# Autodesk Inventor assembly: Asem_Rev2
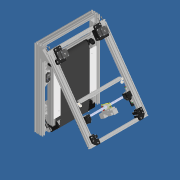
[picture p0: Inventor's stored thumbnail of the model, 180x180]
Saved by Autodesk Inventor 2020 (Build 240168000, 168)
## iProperties
Created: 2020-10-05
Part Number: Asem_Rev2
Document SubType Name: Assembly
Designer: magnarecta
Author: magnarecta
## Documents named in this file (20)
- D:\Document\Github\CoreXY_Laser\Model\Asem\Asem_Rev2.iam
- D:\Document\Github\CoreXY_Laser\Model\Asem\CoreXY_Unit_Asem.iam
- D:\Document\Github\CoreXY_Laser\Model\Parts\MISUMI\HFS5-2060-560_Autodesk_Inventor_2020_20201006\HFS5-2060-560.ipt
- D:\Document\Github\CoreXY_Laser\Model\Asem\Belt_Unit_Asem_Rev3.iam
- D:\Document\Github\CoreXY_Laser\Model\Parts\MISUMI\HFS5-2040-380_Autodesk_Inventor_2020_20201031\HFS5-2040-380.ipt
- D:\Document\Github\CoreXY_Laser\Model\Parts\MISUMI\HBLFSD5-SEC_Autodesk_Inventor_2020_20201031\AIS2020\HBLFSD5-SEC.iam
- D:\Document\Github\CoreXY_Laser\Model\Parts\MISUMI\HBLFSN5-SEC_Autodesk_Inventor_2020_20201031\AIS2020\HBLFSN5-SEC.iam
- D:\Document\Github\CoreXY_Laser\Model\Parts\MISUMI\HBLFSNF5-SEC_Autodesk_Inventor_2020_20201031\AIS2020\HBLFSNF5-SEC_b.iam
- D:\Document\Github\CoreXY_Laser\Model\Parts\Electrical_Components\mean-well-lrs-350-24-1.snapshot.3\meanwell_lrs-350-24_UPDATED.ipt
- D:\Document\Github\CoreXY_Laser\Model\Parts\Electrical_Components\BIGTREETECH_SKR_V1.4\BTT_SKR_V1.4 v13_TOP.iam
- D:\Document\Github\CoreXY_Laser\Model\Parts\Electrical_Components\ac-power-switch-assembly-1.snapshot.2\AC Power Switch Assy.iam
- D:\Document\Github\CoreXY_Laser\Model\Parts\Print_Parts\Rev2_Parts\Print_Parts_L1.ipt
- D:\Document\Github\CoreXY_Laser\Model\Parts\Electrical_Components\biqu-heat-bed-power-module-expansion-hot-bed-mos-tube-for-3d-printer-1.snapshot.2\BIQU-3D0109.iam
- D:\Document\Github\CoreXY_Laser\Model\Parts\Print_Parts\Rev2_Parts\Print_Parts_E2.ipt
- D:\Document\Github\CoreXY_Laser\Model\Parts\Electrical_Components\bigtreetech-tft-24-touchscreen-1.snapshot.2\BIGTREE_TFT24.iam
- D:\Document\Github\CoreXY_Laser\Model\Parts\Print_Parts\Rev2_Parts\Print_Parts_TFT.ipt
- D:\Document\Github\CoreXY_Laser\Model\Parts\Print_Parts\Print_Parts_V.ipt
- D:\Document\Github\CoreXY_Laser\Model\Parts\Print_Parts\Print_Parts_W.ipt
- D:\Document\Github\CoreXY_Laser\Model\Parts\Print_Parts\Print_Model\Controller_Unit\C_Unit_Cable_Holder_A.ipt
- D:\Document\Github\CoreXY_Laser\Model\Parts\Print_Parts\Print_Model\Controller_Unit\C_Unit_Cable_Holder_B.ipt
## Components (36 placed, 19 different names)
1. CoreXY_Unit_Asem:1 [sub-assembly] — フラッシュ:60, メイト:75, メイト:76
2. HFS5-2060-560:1 — フラッシュ:18, フラッシュ:19, Mate:16, Mate:17, Flush:28, Flush:29, Mate:18, Mate:25, Mate:32, Mate:33, Mate:45, Mate:49, Mate:61, メイト:77
3. HFS5-2060-560:2 — フラッシュ:18, フラッシュ:19, メイト:14, Flush:26, Flush:27, Mate:21, Mate:24, Mate:34, Mate:35, Mate:36, Flush:43, Mate:37, Mate:40, Mate:43, Mate:44, フラッシュ:60, フラッシュ:62, メイト:78, メイト:79, フラッシュ:63
4. Belt_Unit_Asem_Rev3:1 [sub-assembly] — メイト:14, Flush:38, Mate:51, Mate:52, Mate:53, Mate:54, Flush:51, Flush:53, Mate:59
5. HFS5-2040-380:1 — Mate:16, Flush:26, Flush:27, Mate:22, Mate:23, Flush:33, Flush:38, Mate:69, 角度:6, フラッシュ:64, メイト:83
6. HFS5-2040-380:2 — Mate:17, Flush:28, Flush:29, Mate:19, Mate:20, Flush:31, Mate:40, メイト:73
7. HBLFSD5-SEC:1 [sub-assembly] — Mate:18, Mate:19, Flush:30
8. HBLFSD5-SEC:2 [sub-assembly] — Mate:20, Mate:21, Flush:30, Flush:31
9. HBLFSD5-SEC:3 [sub-assembly] — Mate:22, Mate:25, Flush:32
10. HBLFSD5-SEC:4 [sub-assembly] — Mate:23, Mate:24, Flush:32, Flush:33
11. HBLFSN5-SEC:1 [sub-assembly] — Mate:33, Flush:40, Mate:50, Flush:49
12. HBLFSN5-SEC:2 [sub-assembly] — Mate:32, Flush:40, Flush:42, Flush:48, Mate:47
13. HBLFSN5-SEC:3 [sub-assembly] — Mate:34, Flush:41, Mate:38, Flush:45, Flush:47
14. HBLFSN5-SEC:4 [sub-assembly] — Mate:35, Flush:41, Flush:42, Mate:39, Flush:46
15. HFS5-2040-380:3 — Mate:36, Flush:43, Flush:44, Mate:38, Flush:45, Mate:41, Mate:48, Mate:50, Mate:56, Mate:57, Mate:59, メイト:73, メイト:84, フラッシュ:65, メイト:91, フラッシュ:67
16. HFS5-2040-380:4 — Mate:37, Flush:44, Mate:39, Mate:42, Mate:46, Mate:47, Mate:55, Mate:58, Mate:69, メイト:87
17. HBLFSN5-SEC:5 [sub-assembly] — Mate:45, Mate:46, Flush:48
18. HBLFSN5-SEC:6 [sub-assembly] — Mate:48, Mate:49, Flush:49
19. HBLFSN5-SEC:7 [sub-assembly] — Mate:41, Mate:43, Flush:47
20. HBLFSN5-SEC:8 [sub-assembly] — Mate:42, Mate:44, Flush:46
21. HBLFSNF5-SEC_b:1 [sub-assembly] — Mate:51, Mate:57, Flush:50, Flush:51
22. HBLFSNF5-SEC_b:2 [sub-assembly] — Mate:52, Mate:58, Flush:50
23. HBLFSNF5-SEC_b:3 [sub-assembly] — Mate:53, Mate:56, Flush:52, Flush:53
24. HBLFSNF5-SEC_b:4 [sub-assembly] — Mate:54, Mate:55, Flush:52
25. AC Power Switch Assy:1 [sub-assembly] — Mate:61, 挿入:3, 挿入:4
26. BIQU-3D0109:1 [sub-assembly] — 挿入:7, メイト:89
27. Print_Parts_L1:4 — メイト:75, メイト:76, フラッシュ:62, メイト:77, メイト:78
28. Print_Parts_E2:1 — メイト:79, フラッシュ:63, 挿入:3, 挿入:4
29. BIGTREE_TFT24:1 [sub-assembly] — メイト:80, メイト:81, メイト:82
30. Print_Parts_TFT:1 — メイト:80, メイト:81, メイト:82, 角度:6, フラッシュ:64, メイト:83
31. Print_Parts_V:1 — メイト:84, フラッシュ:65, メイト:85, 角度:7, 挿入:5, メイト:86, フラッシュ:66
32. meanwell_lrs-350-24_UPDATED:2 — メイト:85, 角度:7, 挿入:5
33. BTT_SKR_V1.4 v13_TOP:2 [sub-assembly] — 挿入:6, メイト:88
34. Print_Parts_W:2 — メイト:86, フラッシュ:66, メイト:87, 挿入:6, メイト:88, 挿入:7, メイト:89
35. C_Unit_Cable_Holder_A:1 — 挿入:8, メイト:92
36. C_Unit_Cable_Holder_B:1 — メイト:91, フラッシュ:67, 挿入:8, メイト:92
## Relationships (99: Mate 59, Flush 32, Insert 6, Angle 2)
- フラッシュ:18 [Flush]: HFS5-2060-560:1 ↔ HFS5-2060-560:2
- フラッシュ:19 [Flush]: HFS5-2060-560:1 ↔ HFS5-2060-560:2
- メイト:14 [Mate] (35 mm): HFS5-2060-560:2 ↔ Belt_Unit_Asem_Rev3:1
- Mate:16: HFS5-2060-560:1 ↔ HFS5-2040-380:1
- Flush:26: HFS5-2060-560:2 ↔ HFS5-2040-380:1
- Flush:27: HFS5-2060-560:2 ↔ HFS5-2040-380:1
- Mate:17: HFS5-2060-560:1 ↔ HFS5-2040-380:2
- Flush:28: HFS5-2060-560:1 ↔ HFS5-2040-380:2
- Flush:29: HFS5-2060-560:1 ↔ HFS5-2040-380:2
- Mate:18: HFS5-2060-560:1 ↔ HBLFSD5-SEC:1
- Mate:19: HFS5-2040-380:2 ↔ HBLFSD5-SEC:1
- Mate:20: HFS5-2040-380:2 ↔ HBLFSD5-SEC:2
- Mate:21: HFS5-2060-560:2 ↔ HBLFSD5-SEC:2
- Flush:30: HBLFSD5-SEC:1 ↔ HBLFSD5-SEC:2
- Flush:31: HFS5-2040-380:2 ↔ HBLFSD5-SEC:2
- Mate:22: HFS5-2040-380:1 ↔ HBLFSD5-SEC:3
- Mate:23: HFS5-2040-380:1 ↔ HBLFSD5-SEC:4
- Mate:24: HFS5-2060-560:2 ↔ HBLFSD5-SEC:4
- Mate:25: HFS5-2060-560:1 ↔ HBLFSD5-SEC:3
- Flush:32: HBLFSD5-SEC:3 ↔ HBLFSD5-SEC:4
- Flush:33: HFS5-2040-380:1 ↔ HBLFSD5-SEC:4
- Flush:38: Belt_Unit_Asem_Rev3:1 ↔ HFS5-2040-380:1
- Mate:32: HFS5-2060-560:1 ↔ HBLFSN5-SEC:2
- Mate:33: HFS5-2060-560:1 ↔ HBLFSN5-SEC:1
- Flush:40: HBLFSN5-SEC:1 ↔ HBLFSN5-SEC:2
- Mate:34: HFS5-2060-560:2 ↔ HBLFSN5-SEC:3
- Mate:35: HFS5-2060-560:2 ↔ HBLFSN5-SEC:4
- Flush:41: HBLFSN5-SEC:3 ↔ HBLFSN5-SEC:4
- Flush:42: HBLFSN5-SEC:2 ↔ HBLFSN5-SEC:4
- Mate:36: HFS5-2060-560:2 ↔ HFS5-2040-380:3
- Flush:43 (20 mm): HFS5-2060-560:2 ↔ HFS5-2040-380:3
- Mate:37: HFS5-2060-560:2 ↔ HFS5-2040-380:4
- Flush:44: HFS5-2040-380:3 ↔ HFS5-2040-380:4
- Mate:38: HBLFSN5-SEC:3 ↔ HFS5-2040-380:3
- Flush:45: HBLFSN5-SEC:3 ↔ HFS5-2040-380:3
- Mate:39: HBLFSN5-SEC:4 ↔ HFS5-2040-380:4
- Mate:40: HFS5-2060-560:2 ↔ HFS5-2040-380:2
- Mate:41: HFS5-2040-380:3 ↔ HBLFSN5-SEC:7
- Mate:42: HFS5-2040-380:4 ↔ HBLFSN5-SEC:8
- Mate:43: HFS5-2060-560:2 ↔ HBLFSN5-SEC:7
- Mate:44: HFS5-2060-560:2 ↔ HBLFSN5-SEC:8
- Flush:46: HBLFSN5-SEC:4 ↔ HBLFSN5-SEC:8
- Flush:47: HBLFSN5-SEC:3 ↔ HBLFSN5-SEC:7
- Mate:45: HFS5-2060-560:1 ↔ HBLFSN5-SEC:5
- Mate:46: HFS5-2040-380:4 ↔ HBLFSN5-SEC:5
- Flush:48: HBLFSN5-SEC:2 ↔ HBLFSN5-SEC:5
- Mate:47: HBLFSN5-SEC:2 ↔ HFS5-2040-380:4
- Mate:48: HFS5-2040-380:3 ↔ HBLFSN5-SEC:6
- Mate:49: HFS5-2060-560:1 ↔ HBLFSN5-SEC:6
- Mate:50: HBLFSN5-SEC:1 ↔ HFS5-2040-380:3
- Flush:49: HBLFSN5-SEC:1 ↔ HBLFSN5-SEC:6
- Mate:51: Belt_Unit_Asem_Rev3:1 ↔ HBLFSNF5-SEC_b:1
- Mate:52: Belt_Unit_Asem_Rev3:1 ↔ HBLFSNF5-SEC_b:2
- Mate:53: Belt_Unit_Asem_Rev3:1 ↔ HBLFSNF5-SEC_b:3
- Mate:54: Belt_Unit_Asem_Rev3:1 ↔ HBLFSNF5-SEC_b:4
- Mate:55: HFS5-2040-380:4 ↔ HBLFSNF5-SEC_b:4
- Mate:56: HFS5-2040-380:3 ↔ HBLFSNF5-SEC_b:3
- Mate:57: HFS5-2040-380:3 ↔ HBLFSNF5-SEC_b:1
- Mate:58: HFS5-2040-380:4 ↔ HBLFSNF5-SEC_b:2
- Flush:50: HBLFSNF5-SEC_b:1 ↔ HBLFSNF5-SEC_b:2
- Flush:51: Belt_Unit_Asem_Rev3:1 ↔ HBLFSNF5-SEC_b:1
- Flush:52: HBLFSNF5-SEC_b:3 ↔ HBLFSNF5-SEC_b:4
- Flush:53: Belt_Unit_Asem_Rev3:1 ↔ HBLFSNF5-SEC_b:3
- Mate:59: Belt_Unit_Asem_Rev3:1 ↔ HFS5-2040-380:3
- Mate:61: HFS5-2060-560:1 ↔ AC Power Switch Assy:1
- Mate:69 (100 mm): HFS5-2040-380:1 ↔ HFS5-2040-380:4
- メイト:73 [Mate] (95 mm): HFS5-2040-380:2 ↔ HFS5-2040-380:3
- フラッシュ:60 [Flush]: CoreXY_Unit_Asem:1 ↔ HFS5-2060-560:2
- メイト:75 [Mate]: CoreXY_Unit_Asem:1 ↔ Print_Parts_L1:4
- メイト:76 [Mate]: CoreXY_Unit_Asem:1 ↔ Print_Parts_L1:4
- フラッシュ:62 [Flush] (-5 mm): HFS5-2060-560:2 ↔ Print_Parts_L1:4
- メイト:77 [Mate]: HFS5-2060-560:1 ↔ Print_Parts_L1:4
- メイト:78 [Mate]: HFS5-2060-560:2 ↔ Print_Parts_L1:4
- メイト:79 [Mate]: HFS5-2060-560:2 ↔ Print_Parts_E2:1
- フラッシュ:63 [Flush]: HFS5-2060-560:2 ↔ Print_Parts_E2:1
- 挿入:3 [Insert]: AC Power Switch Assy:1 ↔ Print_Parts_E2:1
- 挿入:4 [Insert]: AC Power Switch Assy:1 ↔ Print_Parts_E2:1
- メイト:80 [Mate]: BIGTREE_TFT24:1 ↔ Print_Parts_TFT:1
- メイト:81 [Mate]: BIGTREE_TFT24:1 ↔ Print_Parts_TFT:1
- メイト:82 [Mate]: BIGTREE_TFT24:1 ↔ Print_Parts_TFT:1
- 角度:6 [Angle] (45 deg): HFS5-2040-380:1 ↔ Print_Parts_TFT:1
- フラッシュ:64 [Flush]: HFS5-2040-380:1 ↔ Print_Parts_TFT:1
- メイト:83 [Mate]: HFS5-2040-380:1 ↔ Print_Parts_TFT:1
- メイト:84 [Mate]: HFS5-2040-380:3 ↔ Print_Parts_V:1
- フラッシュ:65 [Flush]: HFS5-2040-380:3 ↔ Print_Parts_V:1
- メイト:85 [Mate]: Print_Parts_V:1 ↔ meanwell_lrs-350-24_UPDATED:2
- 角度:7 [Angle] (180 deg): Print_Parts_V:1 ↔ meanwell_lrs-350-24_UPDATED:2
- 挿入:5 [Insert]: Print_Parts_V:1 ↔ meanwell_lrs-350-24_UPDATED:2
- メイト:86 [Mate]: Print_Parts_V:1 ↔ Print_Parts_W:2
- フラッシュ:66 [Flush]: Print_Parts_V:1 ↔ Print_Parts_W:2
- メイト:87 [Mate]: HFS5-2040-380:4 ↔ Print_Parts_W:2
- 挿入:6 [Insert]: BTT_SKR_V1.4 v13_TOP:2 ↔ Print_Parts_W:2
- メイト:88 [Mate]: BTT_SKR_V1.4 v13_TOP:2 ↔ Print_Parts_W:2
- 挿入:7 [Insert]: BIQU-3D0109:1 ↔ Print_Parts_W:2
- メイト:89 [Mate]: BIQU-3D0109:1 ↔ Print_Parts_W:2
- メイト:91 [Mate]: HFS5-2040-380:3 ↔ C_Unit_Cable_Holder_B:1
- フラッシュ:67 [Flush] (-5 mm): HFS5-2040-380:3 ↔ C_Unit_Cable_Holder_B:1
- 挿入:8 [Insert]: C_Unit_Cable_Holder_A:1 ↔ C_Unit_Cable_Holder_B:1
- メイト:92 [Mate]: C_Unit_Cable_Holder_A:1 ↔ C_Unit_Cable_Holder_B:1
